# Autodesk Inventor assembly: Custom_Delta_Assembly
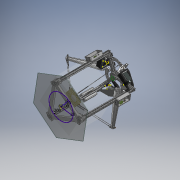
[picture p0: Inventor's stored thumbnail of the model, 180x180]
Saved by Autodesk Inventor 2019.4 (Build 234330000, 330)
## iProperties
Created: 2019-07-06
Part Number: Custom_Delta_Assembly
Document SubType Name: Assembly
Designer: Jorian Brusind
Author: Jorian Brusind
## Documents named in this file (25)
- C:\Users\Jorian Bruslind\Documents\GitHub\ECE44x_Senior_Design\Design files\Delta Robot Arm\Inventor Files\Custom_Delta\Custom_Delta_Assembly.iam
- C:\Users\Jorian Bruslind\Documents\GitHub\ECE44x_Senior_Design\Design files\Delta Robot Arm\Inventor Files\Custom_Delta\Stepper_Face.ipt
- C:\Users\Jorian Bruslind\Documents\GitHub\ECE44x_Senior_Design\Design files\Delta Robot Arm\Inventor Files\Custom_Delta\Delta_Arm.ipt
- C:\Users\Jorian Bruslind\Documents\GitHub\ECE44x_Senior_Design\Design files\Delta Robot Arm\Inventor Files\Custom_Delta\Delta_Top.ipt
- C:\Users\Jorian Bruslind\Documents\GitHub\ECE44x_Senior_Design\Design files\Delta Robot Arm\Inventor Files\McMaster Files\59935K140_METRIC BALL JOINT ROD END.ipt
- C:\Users\Jorian Bruslind\Documents\GitHub\ECE44x_Senior_Design\Design files\PetriFilm\PetriFilm.iam
- C:\Users\Jorian Bruslind\Documents\GitHub\ECE44x_Senior_Design\Design files\Delta Robot Arm\Inventor Files\McMaster Files\5537T501_ALUMINUM T-SLOTTED FRAMING EXTRUSION.ipt
- C:\Users\Jorian Bruslind\Documents\GitHub\ECE44x_Senior_Design\Design files\Delta Robot Arm\Inventor Files\McMaster Files\5537T518_T-SLOTTED FRAMING.ipt
- C:\Users\Jorian Bruslind\Documents\GitHub\ECE44x_Senior_Design\Design files\Delta Robot Arm\Inventor Files\McMaster Files\6In_ALUMINUM T-SLOTTED FRAMING EXTRUSION.ipt
- C:\Users\Jorian Bruslind\Documents\GitHub\ECE44x_Senior_Design\Design files\Delta Robot Arm\Inventor Files\Custom_Delta\80_20_Connector.ipt
- C:\Users\Jorian Bruslind\Documents\GitHub\ECE44x_Senior_Design\Design files\Delta Robot Arm\Inventor Files\Custom_Delta\NEMA17_Stepper_CL42H60.ipt
- C:\Users\Jorian Bruslind\Documents\GitHub\ECE44x_Senior_Design\Design files\Delta Robot Arm\Inventor Files\Stepper_Collar\products\12196\step\model.ipt
- C:\Users\Jorian Bruslind\Documents\GitHub\ECE44x_Senior_Design\Design files\Delta Robot Arm\Inventor Files\raspberry-pi-camera-module-v2-1.snapshot.3\RspCameraMia.iam
- C:\Users\Jorian Bruslind\Documents\GitHub\ECE44x_Senior_Design\Design files\Delta Robot Arm\Inventor Files\Custom_Delta\80_20_Connector_Bot.ipt
- C:\Users\Jorian Bruslind\Documents\GitHub\ECE44x_Senior_Design\Design files\Delta Robot Arm\Inventor Files\endstop-mechanical-limit-switch-on-pcb-1.snapshot.1\Switch.ipt
- C:\Users\Jorian Bruslind\Documents\GitHub\ECE44x_Senior_Design\Design files\Delta Robot Arm\Inventor Files\Custom_Delta\Bottom_Mount.ipt
- C:\Users\Jorian Bruslind\Documents\GitHub\ECE44x_Senior_Design\Design files\Delta Robot Arm\Inventor Files\McMaster Files\98861A050_LOW-STRENGTH STEEL THREADED ROD.ipt
- C:\Users\Jorian Bruslind\Documents\GitHub\ECE44x_Senior_Design\Design files\Delta Robot Arm\Inventor Files\Custom_Delta\Motor_Node.iam
- C:\Users\Jorian Bruslind\Documents\GitHub\ECE44x_Senior_Design\Design files\Delta Robot Arm\Inventor Files\Metric bolt\Bolt M5 20mm.ipt
- C:\Users\Jorian Bruslind\Documents\GitHub\ECE44x_Senior_Design\Design files\Delta Robot Arm\Inventor Files\Custom_Delta\Workarea.ipt
- C:\Users\Jorian Bruslind\Documents\GitHub\ECE44x_Senior_Design\Design files\Delta Robot Arm\Inventor Files\Metric bolt\Bolt M3 50mm.ipt
- C:\Users\Jorian Bruslind\Documents\GitHub\ECE44x_Senior_Design\Design files\Delta Robot Arm\Inventor Files\Custom_Delta\11mmSpacer.ipt
- C:\Users\Jorian Bruslind\Documents\GitHub\ECE44x_Senior_Design\Design files\Delta Robot Arm\Inventor Files\Custom_Delta\5mmSpacer.ipt
- C:\Users\Jorian Bruslind\Documents\GitHub\ECE44x_Senior_Design\Design files\Delta Robot Arm\Inventor Files\Metric nuts\Nut M3.ipt
- C:\Users\Jorian Bruslind\Documents\GitHub\ECE44x_Senior_Design\Design files\Delta Robot Arm\Inventor Files\Custom_Delta\Custom_Delta_End_Effector.ipt
## Components (96 placed, 24 different names)
1. Stepper_Face:1 — Mate:126, Flush:20, Flush:23, Mate:210, Mate:211, Mate:212, Mate:216
2. Delta_Arm:1 — Mate:145, Mate:146, Mate:214, Mate:215, Mate:254, Mate:360, Mate:361, Mate:414
3. Stepper_Face:2 — Mate:125, Flush:18, Flush:24, Mate:222, Mate:227, Mate:230, Mate:231
4. Delta_Arm:2 — Mate:151, Mate:152, Mate:220, Mate:221, Mate:253, Mate:321, Mate:415, Mate:419
5. Stepper_Face:3 — Mate:127, Flush:21, Flush:22, Mate:217, Mate:218, Mate:226, Mate:228
6. Delta_Arm:3 — Mate:224, Mate:225, Mate:229, Mate:333, Mate:341, Mate:345, Mate:346, Mate:439
7. Delta_Top:1 — Mate:103, Mate:105, Mate:106, Mate:107, Mate:109, Mate:110, Mate:111, Mate:112, Mate:113, Mate:189, Mate:190, Mate:191, Mate:192, Mate:238, Mate:240, Mate:241, Mate:243, Mate:244, Mate:246, Mate:411, Mate:470
8. PetriFilm:1 [sub-assembly] — Mate:477
9. 5537T518_T-SLOTTED FRAMING:1 — Mate:106, Mate:107, Mate:119, Flush:30
10. 5537T518_T-SLOTTED FRAMING:2 — Mate:103, Mate:105, Mate:118
11. 5537T518_T-SLOTTED FRAMING:3 — Mate:109, Mate:110, Mate:117
12. 6In_ALUMINUM T-SLOTTED FRAMING EXTRUSION:1 — Flush:5, Mate:121, Flush:6, Mate:126, Flush:20, Flush:23, Mate:188, Mate:235, Mate:247, Mate:412
13. 6In_ALUMINUM T-SLOTTED FRAMING EXTRUSION:2 — Flush:9, Flush:10, Mate:123, Mate:125, Flush:18, Flush:24, Mate:237
14. 6In_ALUMINUM T-SLOTTED FRAMING EXTRUSION:3 — Flush:7, Flush:8, Mate:122, Mate:127, Flush:21, Flush:22, Mate:233
15. 5537T501_ALUMINUM T-SLOTTED FRAMING EXTRUSION:1 — Mate:112, Mate:118, Flush:5, Mate:121, Flush:6, Mate:192, Mate:234, Flush:26, Mate:245, Mate:357, Mate:358, Mate:409, Mate:410, Flush:33
16. 5537T501_ALUMINUM T-SLOTTED FRAMING EXTRUSION:2 — Mate:111, Mate:119, Flush:7, Flush:8, Mate:122, Mate:190, Mate:232, Flush:25, Mate:239, Mate:355, Mate:359, Mate:405, Mate:406, Flush:31
17. 5537T501_ALUMINUM T-SLOTTED FRAMING EXTRUSION:3 — Mate:113, Mate:117, Flush:9, Flush:10, Mate:123, Mate:191, Mate:236, Flush:27, Mate:242, Mate:354, Mate:356, Mate:407, Mate:408, Flush:32
18. 80_20_Connector:1 — Mate:188, Mate:189, Mate:248, Mate:249, Mate:255, Mate:256, Mate:263, Mate:264, Mate:265, Mate:266, Mate:267
19. NEMA17_Stepper_CL42H60:1 — Mate:219, Mate:227, Mate:230, Mate:231
20. NEMA17_Stepper_CL42H60:2 — Mate:210, Mate:211, Mate:212, Mate:213
21. NEMA17_Stepper_CL42H60:3 — Mate:217, Mate:218, Mate:223, Mate:228
22. model:4 — Mate:223, Mate:224, Mate:225, Mate:226, Mate:229
23. model:5 — Mate:213, Mate:214, Mate:215, Mate:216, Mate:254
24. model:6 — Mate:219, Mate:220, Mate:221, Mate:222, Mate:253
25. 5537T518_T-SLOTTED FRAMING:4 — Mate:236, Mate:237, Flush:27
26. 5537T518_T-SLOTTED FRAMING:5 — Mate:232, Mate:233, Flush:25
27. 5537T518_T-SLOTTED FRAMING:6 — Mate:234, Mate:235, Flush:26
28. 5537T518_T-SLOTTED FRAMING:7 — Mate:238, Mate:239, Mate:240, Flush:28
29. 5537T518_T-SLOTTED FRAMING:8 — Mate:241, Mate:242, Mate:243
30. 5537T518_T-SLOTTED FRAMING:9 — Mate:244, Mate:245, Mate:246, Flush:29
31. RspCameraMia:1 [sub-assembly] — Mate:250, Mate:251, Mate:252
32. 80_20_Connector_Bot:1 — Mate:247, Mate:248, Mate:249, Mate:250, Mate:251, Mate:252
33. Switch:1 — Mate:255, Mate:256, Mate:263
34. Switch:2
35. Switch:3
36. 80_20_Connector:2 — Mate:264, Mate:265, Mate:266, Mate:268, Mate:269
37. 80_20_Connector:3 — Mate:267, Mate:268, Mate:269
38. Bottom_Mount:1 — Mate:354, Mate:355, Flush:28
39. Bottom_Mount:3 — Mate:356, Mate:357, Flush:29
40. Bottom_Mount:4 — Mate:358, Mate:359, Flush:30
41. 59935K140_METRIC BALL JOINT ROD END:22 — Mate:333, Mate:346, Mate:380, Mate:382, Mate:443
42. 59935K140_METRIC BALL JOINT ROD END:23 — Mate:341, Mate:345, Mate:377, Mate:379, Mate:413, Mate:437, Mate:441, Mate:445
43. 59935K140_METRIC BALL JOINT ROD END:2 — Mate:145, Mate:146, Mate:390, Mate:391, Mate:432, Mate:434
44. 59935K140_METRIC BALL JOINT ROD END:24 — Mate:360, Mate:361, Mate:385, Mate:386, Mate:428, Mate:430, Mate:436
45. 59935K140_METRIC BALL JOINT ROD END:17 — Mate:321, Mate:370, Mate:372, Mate:419, Mate:423, Mate:425
46. 59935K140_METRIC BALL JOINT ROD END:3 — Mate:151, Mate:152, Mate:374, Mate:416, Mate:421
47. 98861A050_LOW-STRENGTH STEEL THREADED ROD:2 — Mate:369, Mate:370, Mate:371, Mate:372
48. 98861A050_LOW-STRENGTH STEEL THREADED ROD:3 — Mate:376, Mate:377, Mate:378, Mate:379
49. 98861A050_LOW-STRENGTH STEEL THREADED ROD:4 — Mate:380, Mate:382, Mate:383
50. 98861A050_LOW-STRENGTH STEEL THREADED ROD:5 — Mate:373, Mate:374, Mate:375
51. 98861A050_LOW-STRENGTH STEEL THREADED ROD:6 — Mate:384, Mate:385, Mate:386, Mate:387
52. 59935K140_METRIC BALL JOINT ROD END:25 — Mate:376, Mate:378, Mate:472
53. 59935K140_METRIC BALL JOINT ROD END:26 — Mate:369, Mate:371, Mate:475
54. 59935K140_METRIC BALL JOINT ROD END:27 — Mate:384, Mate:387, Mate:474
55. 59935K140_METRIC BALL JOINT ROD END:28 — Mate:373, Mate:375, Mate:476
56. 59935K140_METRIC BALL JOINT ROD END:29 — Mate:389, Mate:473
57. 59935K140_METRIC BALL JOINT ROD END:30 — Mate:383, Mate:471
58. 98861A050_LOW-STRENGTH STEEL THREADED ROD:7 — Mate:389, Mate:390, Mate:391
59. Motor_Node:1 [sub-assembly] — Mate:397, Mate:398, Mate:399, Mate:400, Mate:407, Mate:408, Flush:32
60. Motor_Node:2 [sub-assembly] — Mate:395, Mate:396, Mate:401, Mate:402, Mate:405, Mate:406, Flush:31
61. Motor_Node:3 [sub-assembly] — Mate:393, Mate:394, Mate:403, Mate:404, Mate:409, Mate:410, Flush:33
62. Bolt M5 20mm:1 — Mate:394, Mate:404
63. Bolt M5 20mm:2 — Mate:395, Mate:402
64. Bolt M5 20mm:3 — Mate:396, Mate:401
65. Bolt M5 20mm:4 — Mate:393, Mate:403
66. Bolt M5 20mm:5 — Mate:397, Mate:399
67. Bolt M5 20mm:6 — Mate:398, Mate:400
68. Workarea:1 — Mate:411, Mate:412
69. Bolt M3 50mm:1 — Mate:414, Mate:428, Mate:429, Mate:431, Mate:433, Mate:435, Mate:448
70. Bolt M3 50mm:2 — Mate:415, Mate:416, Mate:420, Mate:422, Mate:424, Mate:426, Mate:427, Mate:450
71. Bolt M3 50mm:3 — Mate:413, Mate:437, Mate:438, Mate:440, Mate:442, Mate:444, Mate:446
72. 11mmSpacer:1 — Mate:420, Mate:421
73. 11mmSpacer:2 — Mate:438, Mate:439
74. 11mmSpacer:3 — Mate:429, Mate:430
75. 11mmSpacer:4 — Mate:422, Mate:423
76. 11mmSpacer:5 — Mate:431, Mate:432
77. 11mmSpacer:6 — Mate:440, Mate:441
78. 5mmSpacer:1 — Mate:433, Mate:434, Mate:449
79. 5mmSpacer:2 — Mate:424, Mate:425, Mate:451
80. 5mmSpacer:3 — Mate:442, Mate:443, Mate:447
81. 5mmSpacer:4 — Mate:444, Mate:445
82. 5mmSpacer:5 — Mate:435, Mate:436
83. 5mmSpacer:6 — Mate:426, Mate:427
84. Nut M3:1 — Mate:450, Mate:451
85. Nut M3:2 — Mate:446, Mate:447
86. Nut M3:3 — Mate:448, Mate:449
87. Custom_Delta_End_Effector:1 — Mate:452, Mate:453, Mate:454, Mate:455, Mate:456, Mate:457, Mate:459, Mate:461, Mate:463, Mate:465, Mate:467, Mate:469, Mate:470, Mate:477
88. 11mmSpacer:7 — Mate:462, Mate:463
89. 11mmSpacer:8 — Mate:468, Mate:469
90. 11mmSpacer:9 — Mate:460, Mate:461
91. 11mmSpacer:10 — Mate:464, Mate:465
92. 11mmSpacer:11 — Mate:466, Mate:467
93. 11mmSpacer:12 — Mate:458, Mate:459
94. Bolt M3 50mm:4 — Mate:454, Mate:457, Mate:466, Mate:468, Mate:473, Mate:474
95. Bolt M3 50mm:5 — Mate:452, Mate:456, Mate:458, Mate:460, Mate:475, Mate:476
96. Bolt M3 50mm:6 — Mate:453, Mate:455, Mate:462, Mate:464, Mate:471, Mate:472
## Relationships (219: Mate 198, Flush 21)
- Mate:103: Delta_Top:1 ↔ 5537T518_T-SLOTTED FRAMING:2
- Mate:105: Delta_Top:1 ↔ 5537T518_T-SLOTTED FRAMING:2
- Mate:106: Delta_Top:1 ↔ 5537T518_T-SLOTTED FRAMING:1
- Mate:107: Delta_Top:1 ↔ 5537T518_T-SLOTTED FRAMING:1
- Mate:109: Delta_Top:1 ↔ 5537T518_T-SLOTTED FRAMING:3
- Mate:110: Delta_Top:1 ↔ 5537T518_T-SLOTTED FRAMING:3
- Mate:111: Delta_Top:1 ↔ 5537T501_ALUMINUM T-SLOTTED FRAMING EXTRUSION:2
- Mate:112: Delta_Top:1 ↔ 5537T501_ALUMINUM T-SLOTTED FRAMING EXTRUSION:1
- Mate:113: Delta_Top:1 ↔ 5537T501_ALUMINUM T-SLOTTED FRAMING EXTRUSION:3
- Mate:117: 5537T518_T-SLOTTED FRAMING:3 ↔ 5537T501_ALUMINUM T-SLOTTED FRAMING EXTRUSION:3
- Mate:118: 5537T518_T-SLOTTED FRAMING:2 ↔ 5537T501_ALUMINUM T-SLOTTED FRAMING EXTRUSION:1
- Mate:119: 5537T518_T-SLOTTED FRAMING:1 ↔ 5537T501_ALUMINUM T-SLOTTED FRAMING EXTRUSION:2
- Flush:5: 6In_ALUMINUM T-SLOTTED FRAMING EXTRUSION:1 ↔ 5537T501_ALUMINUM T-SLOTTED FRAMING EXTRUSION:1
- Mate:121: 6In_ALUMINUM T-SLOTTED FRAMING EXTRUSION:1 ↔ 5537T501_ALUMINUM T-SLOTTED FRAMING EXTRUSION:1
- Flush:6: 6In_ALUMINUM T-SLOTTED FRAMING EXTRUSION:1 ↔ 5537T501_ALUMINUM T-SLOTTED FRAMING EXTRUSION:1
- Flush:7: 6In_ALUMINUM T-SLOTTED FRAMING EXTRUSION:3 ↔ 5537T501_ALUMINUM T-SLOTTED FRAMING EXTRUSION:2
- Flush:8: 6In_ALUMINUM T-SLOTTED FRAMING EXTRUSION:3 ↔ 5537T501_ALUMINUM T-SLOTTED FRAMING EXTRUSION:2
- Mate:122: 6In_ALUMINUM T-SLOTTED FRAMING EXTRUSION:3 ↔ 5537T501_ALUMINUM T-SLOTTED FRAMING EXTRUSION:2
- Flush:9: 6In_ALUMINUM T-SLOTTED FRAMING EXTRUSION:2 ↔ 5537T501_ALUMINUM T-SLOTTED FRAMING EXTRUSION:3
- Flush:10: 6In_ALUMINUM T-SLOTTED FRAMING EXTRUSION:2 ↔ 5537T501_ALUMINUM T-SLOTTED FRAMING EXTRUSION:3
- Mate:123: 6In_ALUMINUM T-SLOTTED FRAMING EXTRUSION:2 ↔ 5537T501_ALUMINUM T-SLOTTED FRAMING EXTRUSION:3
- Mate:125: Stepper_Face:2 ↔ 6In_ALUMINUM T-SLOTTED FRAMING EXTRUSION:2
- Mate:126: Stepper_Face:1 ↔ 6In_ALUMINUM T-SLOTTED FRAMING EXTRUSION:1
- Mate:127: Stepper_Face:3 ↔ 6In_ALUMINUM T-SLOTTED FRAMING EXTRUSION:3
- Mate:145: Delta_Arm:1 ↔ 59935K140_METRIC BALL JOINT ROD END:2
- Mate:146 (9 mm): Delta_Arm:1 ↔ 59935K140_METRIC BALL JOINT ROD END:2
- Mate:151: Delta_Arm:2 ↔ 59935K140_METRIC BALL JOINT ROD END:3
- Mate:152 (9 mm): Delta_Arm:2 ↔ 59935K140_METRIC BALL JOINT ROD END:3
- Flush:18: Stepper_Face:2 ↔ 6In_ALUMINUM T-SLOTTED FRAMING EXTRUSION:2
- Flush:20: Stepper_Face:1 ↔ 6In_ALUMINUM T-SLOTTED FRAMING EXTRUSION:1
- Flush:21: Stepper_Face:3 ↔ 6In_ALUMINUM T-SLOTTED FRAMING EXTRUSION:3
- Flush:22 (112.406 mm): Stepper_Face:3 ↔ 6In_ALUMINUM T-SLOTTED FRAMING EXTRUSION:3
- Flush:23 (112.206 mm): Stepper_Face:1 ↔ 6In_ALUMINUM T-SLOTTED FRAMING EXTRUSION:1
- Flush:24 (112.406 mm): Stepper_Face:2 ↔ 6In_ALUMINUM T-SLOTTED FRAMING EXTRUSION:2
- Mate:188: 6In_ALUMINUM T-SLOTTED FRAMING EXTRUSION:1 ↔ 80_20_Connector:1
- Mate:189: Delta_Top:1 ↔ 80_20_Connector:1
- Mate:190: Delta_Top:1 ↔ 5537T501_ALUMINUM T-SLOTTED FRAMING EXTRUSION:2
- Mate:191: Delta_Top:1 ↔ 5537T501_ALUMINUM T-SLOTTED FRAMING EXTRUSION:3
- Mate:192: Delta_Top:1 ↔ 5537T501_ALUMINUM T-SLOTTED FRAMING EXTRUSION:1
- Mate:210: Stepper_Face:1 ↔ NEMA17_Stepper_CL42H60:2
- Mate:211: Stepper_Face:1 ↔ NEMA17_Stepper_CL42H60:2
- Mate:212: Stepper_Face:1 ↔ NEMA17_Stepper_CL42H60:2
- Mate:213: NEMA17_Stepper_CL42H60:2 ↔ model:5
- Mate:214: Delta_Arm:1 ↔ model:5
- Mate:215: Delta_Arm:1 ↔ model:5
- Mate:216: Stepper_Face:1 ↔ model:5
- Mate:217: Stepper_Face:3 ↔ NEMA17_Stepper_CL42H60:3
- Mate:218: Stepper_Face:3 ↔ NEMA17_Stepper_CL42H60:3
- Mate:219: NEMA17_Stepper_CL42H60:1 ↔ model:6
- Mate:220: Delta_Arm:2 ↔ model:6
- Mate:221: Delta_Arm:2 ↔ model:6
- Mate:222: Stepper_Face:2 ↔ model:6
- Mate:223: NEMA17_Stepper_CL42H60:3 ↔ model:4
- Mate:224: Delta_Arm:3 ↔ model:4
- Mate:225: Delta_Arm:3 ↔ model:4
- Mate:226: Stepper_Face:3 ↔ model:4
- Mate:227: Stepper_Face:2 ↔ NEMA17_Stepper_CL42H60:1
- Mate:228: Stepper_Face:3 ↔ NEMA17_Stepper_CL42H60:3
- Mate:229: Delta_Arm:3 ↔ model:4
- Mate:230: Stepper_Face:2 ↔ NEMA17_Stepper_CL42H60:1
- Mate:231: Stepper_Face:2 ↔ NEMA17_Stepper_CL42H60:1
- Mate:232: 5537T501_ALUMINUM T-SLOTTED FRAMING EXTRUSION:2 ↔ 5537T518_T-SLOTTED FRAMING:5
- Mate:233: 6In_ALUMINUM T-SLOTTED FRAMING EXTRUSION:3 ↔ 5537T518_T-SLOTTED FRAMING:5
- Flush:25: 5537T501_ALUMINUM T-SLOTTED FRAMING EXTRUSION:2 ↔ 5537T518_T-SLOTTED FRAMING:5
- Mate:234: 5537T501_ALUMINUM T-SLOTTED FRAMING EXTRUSION:1 ↔ 5537T518_T-SLOTTED FRAMING:6
- Mate:235: 6In_ALUMINUM T-SLOTTED FRAMING EXTRUSION:1 ↔ 5537T518_T-SLOTTED FRAMING:6
- Flush:26: 5537T501_ALUMINUM T-SLOTTED FRAMING EXTRUSION:1 ↔ 5537T518_T-SLOTTED FRAMING:6
- Mate:236: 5537T501_ALUMINUM T-SLOTTED FRAMING EXTRUSION:3 ↔ 5537T518_T-SLOTTED FRAMING:4
- Mate:237: 6In_ALUMINUM T-SLOTTED FRAMING EXTRUSION:2 ↔ 5537T518_T-SLOTTED FRAMING:4
- Flush:27: 5537T501_ALUMINUM T-SLOTTED FRAMING EXTRUSION:3 ↔ 5537T518_T-SLOTTED FRAMING:4
- Mate:238: Delta_Top:1 ↔ 5537T518_T-SLOTTED FRAMING:7
- Mate:239: 5537T501_ALUMINUM T-SLOTTED FRAMING EXTRUSION:2 ↔ 5537T518_T-SLOTTED FRAMING:7
- Mate:240: Delta_Top:1 ↔ 5537T518_T-SLOTTED FRAMING:7
- Mate:241: Delta_Top:1 ↔ 5537T518_T-SLOTTED FRAMING:8
- Mate:242: 5537T501_ALUMINUM T-SLOTTED FRAMING EXTRUSION:3 ↔ 5537T518_T-SLOTTED FRAMING:8
- Mate:243: Delta_Top:1 ↔ 5537T518_T-SLOTTED FRAMING:8
- Mate:244: Delta_Top:1 ↔ 5537T518_T-SLOTTED FRAMING:9
- Mate:245: 5537T501_ALUMINUM T-SLOTTED FRAMING EXTRUSION:1 ↔ 5537T518_T-SLOTTED FRAMING:9
- Mate:246: Delta_Top:1 ↔ 5537T518_T-SLOTTED FRAMING:9
- Mate:247: 6In_ALUMINUM T-SLOTTED FRAMING EXTRUSION:1 ↔ 80_20_Connector_Bot:1
- Mate:248: 80_20_Connector:1 ↔ 80_20_Connector_Bot:1
- Mate:249: 80_20_Connector:1 ↔ 80_20_Connector_Bot:1
- Mate:250: RspCameraMia:1 ↔ 80_20_Connector_Bot:1
- Mate:251: RspCameraMia:1 ↔ 80_20_Connector_Bot:1
- Mate:252: RspCameraMia:1 ↔ 80_20_Connector_Bot:1
- Mate:253: Delta_Arm:2 ↔ model:6
- Mate:254: Delta_Arm:1 ↔ model:5
- Mate:255: 80_20_Connector:1 ↔ Switch:1
- Mate:256: 80_20_Connector:1 ↔ Switch:1
- Mate:263: 80_20_Connector:1 ↔ Switch:1
- Mate:264: 80_20_Connector:1 ↔ 80_20_Connector:2
- Mate:265: 80_20_Connector:1 ↔ 80_20_Connector:2
- Mate:266: 80_20_Connector:1 ↔ 80_20_Connector:2
- Mate:267: 80_20_Connector:1 ↔ 80_20_Connector:3
- Mate:268: 80_20_Connector:2 ↔ 80_20_Connector:3
- Mate:269: 80_20_Connector:2 ↔ 80_20_Connector:3
- Mate:321 (9 mm): Delta_Arm:2 ↔ 59935K140_METRIC BALL JOINT ROD END:17
- Mate:333: Delta_Arm:3 ↔ 59935K140_METRIC BALL JOINT ROD END:22
- Mate:341: Delta_Arm:3 ↔ 59935K140_METRIC BALL JOINT ROD END:23
- Mate:345 (9 mm): Delta_Arm:3 ↔ 59935K140_METRIC BALL JOINT ROD END:23
- Mate:346 (9 mm): Delta_Arm:3 ↔ 59935K140_METRIC BALL JOINT ROD END:22
- Mate:354: 5537T501_ALUMINUM T-SLOTTED FRAMING EXTRUSION:3 ↔ Bottom_Mount:1
- Mate:355: 5537T501_ALUMINUM T-SLOTTED FRAMING EXTRUSION:2 ↔ Bottom_Mount:1
- Flush:28: 5537T518_T-SLOTTED FRAMING:7 ↔ Bottom_Mount:1
- Mate:356: 5537T501_ALUMINUM T-SLOTTED FRAMING EXTRUSION:3 ↔ Bottom_Mount:3
- Mate:357: 5537T501_ALUMINUM T-SLOTTED FRAMING EXTRUSION:1 ↔ Bottom_Mount:3
- Flush:29: 5537T518_T-SLOTTED FRAMING:9 ↔ Bottom_Mount:3
- Mate:358: 5537T501_ALUMINUM T-SLOTTED FRAMING EXTRUSION:1 ↔ Bottom_Mount:4
- Mate:359: 5537T501_ALUMINUM T-SLOTTED FRAMING EXTRUSION:2 ↔ Bottom_Mount:4
- Flush:30: 5537T518_T-SLOTTED FRAMING:1 ↔ Bottom_Mount:4
- Mate:360: Delta_Arm:1 ↔ 59935K140_METRIC BALL JOINT ROD END:24
- Mate:361 (9 mm): Delta_Arm:1 ↔ 59935K140_METRIC BALL JOINT ROD END:24
- Mate:369: 98861A050_LOW-STRENGTH STEEL THREADED ROD:2 ↔ 59935K140_METRIC BALL JOINT ROD END:26
- Mate:370: 59935K140_METRIC BALL JOINT ROD END:17 ↔ 98861A050_LOW-STRENGTH STEEL THREADED ROD:2
- Mate:371: 98861A050_LOW-STRENGTH STEEL THREADED ROD:2 ↔ 59935K140_METRIC BALL JOINT ROD END:26
- Mate:372: 59935K140_METRIC BALL JOINT ROD END:17 ↔ 98861A050_LOW-STRENGTH STEEL THREADED ROD:2
- Mate:373: 98861A050_LOW-STRENGTH STEEL THREADED ROD:5 ↔ 59935K140_METRIC BALL JOINT ROD END:28
- Mate:374: 59935K140_METRIC BALL JOINT ROD END:3 ↔ 98861A050_LOW-STRENGTH STEEL THREADED ROD:5
- Mate:375: 98861A050_LOW-STRENGTH STEEL THREADED ROD:5 ↔ 59935K140_METRIC BALL JOINT ROD END:28
- Mate:376: 98861A050_LOW-STRENGTH STEEL THREADED ROD:3 ↔ 59935K140_METRIC BALL JOINT ROD END:25
- Mate:377: 59935K140_METRIC BALL JOINT ROD END:23 ↔ 98861A050_LOW-STRENGTH STEEL THREADED ROD:3
- Mate:378: 98861A050_LOW-STRENGTH STEEL THREADED ROD:3 ↔ 59935K140_METRIC BALL JOINT ROD END:25
- Mate:379: 59935K140_METRIC BALL JOINT ROD END:23 ↔ 98861A050_LOW-STRENGTH STEEL THREADED ROD:3
- Mate:380: 59935K140_METRIC BALL JOINT ROD END:22 ↔ 98861A050_LOW-STRENGTH STEEL THREADED ROD:4
- Mate:382: 59935K140_METRIC BALL JOINT ROD END:22 ↔ 98861A050_LOW-STRENGTH STEEL THREADED ROD:4
- Mate:383: 98861A050_LOW-STRENGTH STEEL THREADED ROD:4 ↔ 59935K140_METRIC BALL JOINT ROD END:30
- Mate:384: 98861A050_LOW-STRENGTH STEEL THREADED ROD:6 ↔ 59935K140_METRIC BALL JOINT ROD END:27
- Mate:385: 59935K140_METRIC BALL JOINT ROD END:24 ↔ 98861A050_LOW-STRENGTH STEEL THREADED ROD:6
- Mate:386: 59935K140_METRIC BALL JOINT ROD END:24 ↔ 98861A050_LOW-STRENGTH STEEL THREADED ROD:6
- Mate:387: 98861A050_LOW-STRENGTH STEEL THREADED ROD:6 ↔ 59935K140_METRIC BALL JOINT ROD END:27
- Mate:389: 59935K140_METRIC BALL JOINT ROD END:29 ↔ 98861A050_LOW-STRENGTH STEEL THREADED ROD:7
- Mate:390: 59935K140_METRIC BALL JOINT ROD END:2 ↔ 98861A050_LOW-STRENGTH STEEL THREADED ROD:7
- Mate:391: 59935K140_METRIC BALL JOINT ROD END:2 ↔ 98861A050_LOW-STRENGTH STEEL THREADED ROD:7
- Mate:393: Motor_Node:3 ↔ Bolt M5 20mm:4
- Mate:394: Motor_Node:3 ↔ Bolt M5 20mm:1
- Mate:395: Motor_Node:2 ↔ Bolt M5 20mm:2
- Mate:396: Motor_Node:2 ↔ Bolt M5 20mm:3
- Mate:397: Motor_Node:1 ↔ Bolt M5 20mm:5
- Mate:398: Motor_Node:1 ↔ Bolt M5 20mm:6
- Mate:399: Motor_Node:1 ↔ Bolt M5 20mm:5
- Mate:400: Motor_Node:1 ↔ Bolt M5 20mm:6
- Mate:401: Motor_Node:2 ↔ Bolt M5 20mm:3
- Mate:402: Motor_Node:2 ↔ Bolt M5 20mm:2
- Mate:403: Motor_Node:3 ↔ Bolt M5 20mm:4
- Mate:404: Motor_Node:3 ↔ Bolt M5 20mm:1
- Mate:405: 5537T501_ALUMINUM T-SLOTTED FRAMING EXTRUSION:2 ↔ Motor_Node:2
- Mate:406 (-35 mm): 5537T501_ALUMINUM T-SLOTTED FRAMING EXTRUSION:2 ↔ Motor_Node:2
- Flush:31 (50 mm): 5537T501_ALUMINUM T-SLOTTED FRAMING EXTRUSION:2 ↔ Motor_Node:2
- Mate:407: 5537T501_ALUMINUM T-SLOTTED FRAMING EXTRUSION:3 ↔ Motor_Node:1
- Mate:408 (-35 mm): 5537T501_ALUMINUM T-SLOTTED FRAMING EXTRUSION:3 ↔ Motor_Node:1
- Flush:32 (50 mm): 5537T501_ALUMINUM T-SLOTTED FRAMING EXTRUSION:3 ↔ Motor_Node:1
- Mate:409: 5537T501_ALUMINUM T-SLOTTED FRAMING EXTRUSION:1 ↔ Motor_Node:3
- Mate:410 (-35 mm): 5537T501_ALUMINUM T-SLOTTED FRAMING EXTRUSION:1 ↔ Motor_Node:3
- Flush:33 (50 mm): 5537T501_ALUMINUM T-SLOTTED FRAMING EXTRUSION:1 ↔ Motor_Node:3
- Mate:411: Delta_Top:1 ↔ Workarea:1
- Mate:412 (160.27 mm): 6In_ALUMINUM T-SLOTTED FRAMING EXTRUSION:1 ↔ Workarea:1
- Mate:413: 59935K140_METRIC BALL JOINT ROD END:23 ↔ Bolt M3 50mm:3
- Mate:414: Delta_Arm:1 ↔ Bolt M3 50mm:1
- Mate:415: Delta_Arm:2 ↔ Bolt M3 50mm:2
- Mate:416 (5 mm): 59935K140_METRIC BALL JOINT ROD END:3 ↔ Bolt M3 50mm:2
- Mate:419: Delta_Arm:2 ↔ 59935K140_METRIC BALL JOINT ROD END:17
- Mate:420: Bolt M3 50mm:2 ↔ 11mmSpacer:1
- Mate:421: 59935K140_METRIC BALL JOINT ROD END:3 ↔ 11mmSpacer:1
- Mate:422: Bolt M3 50mm:2 ↔ 11mmSpacer:4
- Mate:423: 59935K140_METRIC BALL JOINT ROD END:17 ↔ 11mmSpacer:4
- Mate:424: Bolt M3 50mm:2 ↔ 5mmSpacer:2
- Mate:425: 59935K140_METRIC BALL JOINT ROD END:17 ↔ 5mmSpacer:2
- Mate:426: Bolt M3 50mm:2 ↔ 5mmSpacer:6
- Mate:427: Bolt M3 50mm:2 ↔ 5mmSpacer:6
- Mate:428 (5 mm): 59935K140_METRIC BALL JOINT ROD END:24 ↔ Bolt M3 50mm:1
- Mate:429: Bolt M3 50mm:1 ↔ 11mmSpacer:3
- Mate:430: 59935K140_METRIC BALL JOINT ROD END:24 ↔ 11mmSpacer:3
- Mate:431: Bolt M3 50mm:1 ↔ 11mmSpacer:5
- Mate:432: 59935K140_METRIC BALL JOINT ROD END:2 ↔ 11mmSpacer:5
- Mate:433: Bolt M3 50mm:1 ↔ 5mmSpacer:1
- Mate:434: 59935K140_METRIC BALL JOINT ROD END:2 ↔ 5mmSpacer:1
- Mate:435: Bolt M3 50mm:1 ↔ 5mmSpacer:5
- Mate:436: 59935K140_METRIC BALL JOINT ROD END:24 ↔ 5mmSpacer:5
- Mate:437 (5 mm): 59935K140_METRIC BALL JOINT ROD END:23 ↔ Bolt M3 50mm:3
- Mate:438: Bolt M3 50mm:3 ↔ 11mmSpacer:2
- Mate:439: Delta_Arm:3 ↔ 11mmSpacer:2
- Mate:440: Bolt M3 50mm:3 ↔ 11mmSpacer:6
- Mate:441: 59935K140_METRIC BALL JOINT ROD END:23 ↔ 11mmSpacer:6
- Mate:442: Bolt M3 50mm:3 ↔ 5mmSpacer:3
- Mate:443: 59935K140_METRIC BALL JOINT ROD END:22 ↔ 5mmSpacer:3
- Mate:444: Bolt M3 50mm:3 ↔ 5mmSpacer:4
- Mate:445: 59935K140_METRIC BALL JOINT ROD END:23 ↔ 5mmSpacer:4
- Mate:446: Bolt M3 50mm:3 ↔ Nut M3:2
- Mate:447: 5mmSpacer:3 ↔ Nut M3:2
- Mate:448: Bolt M3 50mm:1 ↔ Nut M3:3
- Mate:449: 5mmSpacer:1 ↔ Nut M3:3
- Mate:450: Bolt M3 50mm:2 ↔ Nut M3:1
- Mate:451: 5mmSpacer:2 ↔ Nut M3:1
- Mate:452: Custom_Delta_End_Effector:1 ↔ Bolt M3 50mm:5
- Mate:453: Custom_Delta_End_Effector:1 ↔ Bolt M3 50mm:6
- Mate:454: Custom_Delta_End_Effector:1 ↔ Bolt M3 50mm:4
- Mate:455 (20 mm): Custom_Delta_End_Effector:1 ↔ Bolt M3 50mm:6
- Mate:456 (20 mm): Custom_Delta_End_Effector:1 ↔ Bolt M3 50mm:5
- Mate:457 (20 mm): Custom_Delta_End_Effector:1 ↔ Bolt M3 50mm:4
- Mate:458: 11mmSpacer:12 ↔ Bolt M3 50mm:5
- Mate:459: Custom_Delta_End_Effector:1 ↔ 11mmSpacer:12
- Mate:460: 11mmSpacer:9 ↔ Bolt M3 50mm:5
- Mate:461: Custom_Delta_End_Effector:1 ↔ 11mmSpacer:9
- Mate:462: 11mmSpacer:7 ↔ Bolt M3 50mm:6
- Mate:463: Custom_Delta_End_Effector:1 ↔ 11mmSpacer:7
- Mate:464: 11mmSpacer:10 ↔ Bolt M3 50mm:6
- Mate:465: Custom_Delta_End_Effector:1 ↔ 11mmSpacer:10
- Mate:466: 11mmSpacer:11 ↔ Bolt M3 50mm:4
- Mate:467: Custom_Delta_End_Effector:1 ↔ 11mmSpacer:11
- Mate:468: 11mmSpacer:8 ↔ Bolt M3 50mm:4
- Mate:469: Custom_Delta_End_Effector:1 ↔ 11mmSpacer:8
- Mate:470: Delta_Top:1 ↔ Custom_Delta_End_Effector:1
- Mate:471: 59935K140_METRIC BALL JOINT ROD END:30 ↔ Bolt M3 50mm:6
- Mate:472: 59935K140_METRIC BALL JOINT ROD END:25 ↔ Bolt M3 50mm:6
- Mate:473: 59935K140_METRIC BALL JOINT ROD END:29 ↔ Bolt M3 50mm:4
- Mate:474: 59935K140_METRIC BALL JOINT ROD END:27 ↔ Bolt M3 50mm:4
- Mate:475: 59935K140_METRIC BALL JOINT ROD END:26 ↔ Bolt M3 50mm:5
- Mate:476: 59935K140_METRIC BALL JOINT ROD END:28 ↔ Bolt M3 50mm:5
- Mate:477: PetriFilm:1 ↔ Custom_Delta_End_Effector:1
